# Autodesk Inventor assembly: PCBsUnit
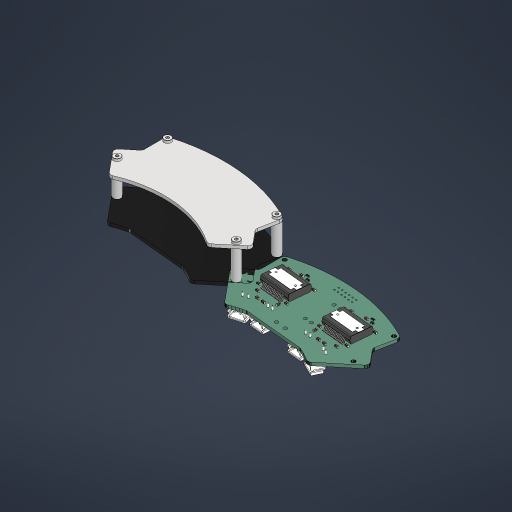
[picture p0: Inventor's stored thumbnail of the model, 512x512]
Saved by Autodesk Inventor 2024.2 (Build 282272000, 272)
## iProperties
Created: 2023-12-28
Part Number: PCBsUnit
Document SubType Name: Assembly
Designer: Hanaoka
Author: Hanaoka
## Documents named in this file (7)
- G:\共有ドライブ\reRo\05_個人\hanaoka\inventor\PCBs\PCBsUnit.iam
- G:\共有ドライブ\reRo\05_個人\hanaoka\inventor\PCBs\MotorDriver_v2\MotorDriver_v2.iam
- G:\共有ドライブ\reRo\05_個人\hanaoka\inventor\Spacer\Spacer_M2x8.ipt
- G:\共有ドライブ\reRo\05_個人\hanaoka\inventor\PCBs\MainMCU_PCB.ipt
- G:\共有ドライブ\reRo\05_個人\hanaoka\inventor\PCBs\MotorDriver_PCB.ipt
- G:\共有ドライブ\reRo\05_個人\hanaoka\inventor\Spacer\Spacer_M2x15.ipt
- G:\共有ドライブ\reRo\05_個人\hanaoka\inventor\Screw\M2xL6\M2x6.ipt
## Components (19 placed, 6 different names)
1. MotorDriver_v2:1 [sub-assembly]
2. Spacer_M2x8:1 — 挿入:2, 挿入:13
3. Spacer_M2x8:2 — 挿入:1, 挿入:12
4. Spacer_M2x8:3 — 挿入:4, 挿入:14
5. Spacer_M2x8:4 — 挿入:3, 挿入:11
6. MainMCU_PCB:1 — 挿入:1, 挿入:2, 挿入:3, 挿入:4, 挿入:5, 挿入:6, 挿入:7, 挿入:8, メイト:2, メイト:3, 正接:1
7. MotorDriver_PCB:1 — 挿入:9, 挿入:10, 挿入:15, 挿入:16, 挿入:17, 挿入:18
8. Spacer_M2x15:1 — 挿入:5, 挿入:10
9. Spacer_M2x15:2 — 挿入:8, 挿入:9
10. Spacer_M2x15:3 — 挿入:6
11. Spacer_M2x15:4 — 挿入:7
12. M2x6:1 — 挿入:18
13. M2x6:2 — 挿入:13
14. M2x6:3 — 挿入:11
15. M2x6:4 — 挿入:17
16. M2x6:5 — 挿入:12
17. M2x6:6 — 挿入:14
18. M2x6:7 — 挿入:16
19. M2x6:8 — 挿入:15
## Relationships (21: Insert 18, Mate 2, Tangent 1)
- 挿入:1 [Insert]: Spacer_M2x8:2 ↔ MainMCU_PCB:1
- 挿入:2 [Insert]: Spacer_M2x8:1 ↔ MainMCU_PCB:1
- 挿入:3 [Insert]: Spacer_M2x8:4 ↔ MainMCU_PCB:1
- 挿入:4 [Insert]: Spacer_M2x8:3 ↔ MainMCU_PCB:1
- 挿入:5 [Insert]: MainMCU_PCB:1 ↔ Spacer_M2x15:1
- 挿入:6 [Insert]: MainMCU_PCB:1 ↔ Spacer_M2x15:3
- 挿入:7 [Insert]: MainMCU_PCB:1 ↔ Spacer_M2x15:4
- 挿入:8 [Insert]: MainMCU_PCB:1 ↔ Spacer_M2x15:2
- 挿入:9 [Insert]: MotorDriver_PCB:1 ↔ Spacer_M2x15:2
- 挿入:10 [Insert]: MotorDriver_PCB:1 ↔ Spacer_M2x15:1
- 挿入:11 [Insert] (1 mm): Spacer_M2x8:4 ↔ M2x6:3
- 挿入:12 [Insert] (1 mm): Spacer_M2x8:2 ↔ M2x6:5
- 挿入:13 [Insert] (1 mm): Spacer_M2x8:1 ↔ M2x6:2
- 挿入:14 [Insert] (1 mm): Spacer_M2x8:3 ↔ M2x6:6
- 挿入:15 [Insert]: MotorDriver_PCB:1 ↔ M2x6:8
- 挿入:16 [Insert]: MotorDriver_PCB:1 ↔ M2x6:7
- 挿入:17 [Insert]: MotorDriver_PCB:1 ↔ M2x6:4
- 挿入:18 [Insert]: MotorDriver_PCB:1 ↔ M2x6:1
- メイト:2 [Mate]: MainMCU_PCB:1
- メイト:3 [Mate]: MainMCU_PCB:1
- 正接:1 [Tangent]: MainMCU_PCB:1
